# Autodesk Inventor assembly: Pump_V3
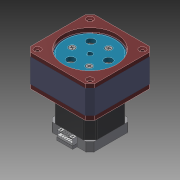
[picture p0: Inventor's stored thumbnail of the model, 180x180]
Saved by Autodesk Inventor 2022 (Build 260153000, 153)
## iProperties
Created: 2025-01-26
Part Number: Pump_V3
Document SubType Name: Assembly
Designer: Ivan
Author: Ivan
## Documents named in this file (11)
- E:\4. Прочее\1517\Предпрофессиональная олимпиада\Насос\Itteration_4\Pump_V3.iam
- E:\4. Прочее\1517\Предпрофессиональная олимпиада\Насос\Itteration_4\Nema_17.ipt
- E:\4. Прочее\1517\Предпрофессиональная олимпиада\Насос\Itteration_4\Pump_V3_Основание.ipt
- E:\4. Прочее\1517\Предпрофессиональная олимпиада\Насос\Itteration_4\ISO 7046-1 - M3 x 8_ - 4.8 - H - ISO.ipt
- E:\4. Прочее\1517\Предпрофессиональная олимпиада\Насос\Itteration_4\Pump_V3_Полумуфта.ipt
- E:\4. Прочее\1517\Предпрофессиональная олимпиада\Насос\Itteration_4\Abec 7 608 zz.ipt
- E:\4. Прочее\1517\Предпрофессиональная олимпиада\Насос\Itteration_4\Pump_V3_Втулка.ipt
- E:\4. Прочее\1517\Предпрофессиональная олимпиада\Насос\Itteration_4\Втулка Впаиваемая М3х4.2х5.ipt
- E:\4. Прочее\1517\Предпрофессиональная олимпиада\Насос\Itteration_4\ISO 7046-1 - M3 x 20_ - 4.8 - H - ISO.ipt
- E:\4. Прочее\1517\Предпрофессиональная олимпиада\Насос\Itteration_4\Pump_V3_Корпус.iam
- E:\4. Прочее\1517\Предпрофессиональная олимпиада\Насос\Itteration_4\Крышка.ipt
## Components (24 placed, 10 different names)
1. Nema_17:1 — Совмещение:1, Совмещение:2, Совмещение:3, Совмещение:5
2. Pump_V3_Основание:1 — Совмещение:1, Совмещение:2, Совмещение:3, Совмещение:4, Заподлицо:1, Совмещение:6, Совмещение:15, Совмещение:16, Совмещение:17
3. Pump_V3_Полумуфта:1 — Совмещение:5, Совмещение:6, Совмещение:7, Совмещение:8, Совмещение:9, Совмещение:10, Совмещение:13, Заподлицо:2, Совмещение:14, Заподлицо:3
4. Pump_V3_Корпус:2 [sub-assembly] — Совмещение:15, Совмещение:16, Совмещение:17, Совмещение:18, Совмещение:19, Совмещение:20
5. Крышка:1 — Совмещение:18, Совмещение:19, Совмещение:20
6. ISO 7046-1 H M3 x 8 - 4.8 - H:2 — Совмещение:4, Заподлицо:1
7. ISO 7046-1 H M3 x 8 - 4.8 - H:3
8. ISO 7046-1 H M3 x 8 - 4.8 - H:4
9. ISO 7046-1 H M3 x 8 - 4.8 - H:5
10. Abec 7 608 zz:1 — Совмещение:7, Совмещение:10, Совмещение:11
11. Abec 7 608 zz:2 — Совмещение:8, Совмещение:9, Совмещение:12
12. Pump_V3_Втулка:1 — Совмещение:11, Совмещение:12
13. Abec 7 608 zz:3
14. Abec 7 608 zz:4
15. Pump_V3_Втулка:2
16. Abec 7 608 zz:5
17. Abec 7 608 zz:6
18. Pump_V3_Втулка:3
19. Втулка Впаиваемая М3х4.2х5:1 — Совмещение:13, Заподлицо:2
20. ISO 7046-1 H M3 x 20 - 4.8 - H:2 — Совмещение:14, Заподлицо:3
21. Втулка Впаиваемая М3х4.2х5:2
22. ISO 7046-1 H M3 x 20 - 4.8 - H:3
23. Втулка Впаиваемая М3х4.2х5:3
24. ISO 7046-1 H M3 x 20 - 4.8 - H:4
## Component patterns: (4 elements, first: ISO 7046-1 H M3 x 8 - 4.8 - H:2), (3 elements, first: Abec 7 608 zz:1 + Abec 7 608 zz:2 + Pump_V3_Втулка:1), (3 elements, first: Втулка Впаиваемая М3х4.2х5:1 + ISO 7046-1 H M3 x 20 - 4.8 - H:2)
## Relationships (23: Mate 20, Flush 3)
- Совмещение:1 [Mate]: Nema_17:1 ↔ Pump_V3_Основание:1
- Совмещение:2 [Mate]: Nema_17:1 ↔ Pump_V3_Основание:1
- Совмещение:3 [Mate]: Nema_17:1 ↔ Pump_V3_Основание:1
- Совмещение:4 [Mate]: Pump_V3_Основание:1 ↔ ISO 7046-1 H M3 x 8 - 4.8 - H:2
- Заподлицо:1 [Flush]: Pump_V3_Основание:1 ↔ ISO 7046-1 H M3 x 8 - 4.8 - H:2
- Совмещение:5 [Mate]: Nema_17:1 ↔ Pump_V3_Полумуфта:1
- Совмещение:6 [Mate]: Pump_V3_Основание:1 ↔ Pump_V3_Полумуфта:1
- Совмещение:7 [Mate]: Pump_V3_Полумуфта:1 ↔ Abec 7 608 zz:1
- Совмещение:8 [Mate]: Pump_V3_Полумуфта:1 ↔ Abec 7 608 zz:2
- Совмещение:9 [Mate]: Pump_V3_Полумуфта:1 ↔ Abec 7 608 zz:2
- Совмещение:10 [Mate]: Pump_V3_Полумуфта:1 ↔ Abec 7 608 zz:1
- Совмещение:11 [Mate]: Abec 7 608 zz:1 ↔ Pump_V3_Втулка:1
- Совмещение:12 [Mate]: Abec 7 608 zz:2 ↔ Pump_V3_Втулка:1
- Совмещение:13 [Mate]: Pump_V3_Полумуфта:1 ↔ Втулка Впаиваемая М3х4.2х5:1
- Заподлицо:2 [Flush]: Pump_V3_Полумуфта:1 ↔ Втулка Впаиваемая М3х4.2х5:1
- Совмещение:14 [Mate]: Pump_V3_Полумуфта:1 ↔ ISO 7046-1 H M3 x 20 - 4.8 - H:2
- Заподлицо:3 [Flush]: Pump_V3_Полумуфта:1 ↔ ISO 7046-1 H M3 x 20 - 4.8 - H:2
- Совмещение:15 [Mate]: Pump_V3_Основание:1 ↔ Pump_V3_Корпус:2
- Совмещение:16 [Mate]: Pump_V3_Основание:1 ↔ Pump_V3_Корпус:2
- Совмещение:17 [Mate]: Pump_V3_Основание:1 ↔ Pump_V3_Корпус:2
- Совмещение:18 [Mate]: Pump_V3_Корпус:2 ↔ Крышка:1
- Совмещение:19 [Mate]: Pump_V3_Корпус:2 ↔ Крышка:1
- Совмещение:20 [Mate]: Pump_V3_Корпус:2 ↔ Крышка:1
